# Autodesk Inventor assembly: Assieme
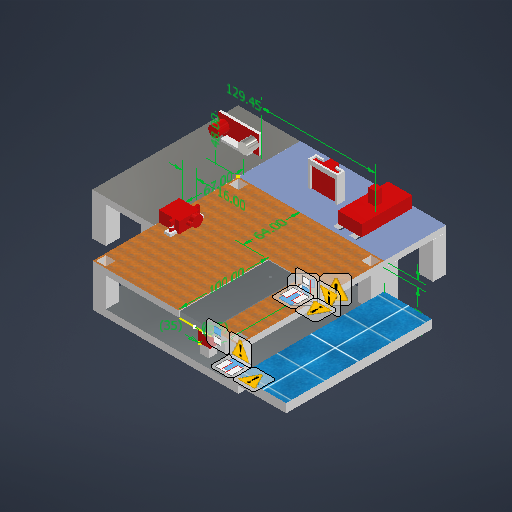
[picture p0: Inventor's stored thumbnail of the model, 512x512]
Saved by Autodesk Inventor 2026.2 (Build 302298000, 298)
## iProperties
Created: 2026-01-19
Part Number: Assieme
Document SubType Name: Assembly
Designer: ASUS
Mass: 649.981 g
Surface Area: 2252.42 cm^2
Volume: 649.981 cm^3
Density: 1 g/cm^3
Author: ASUS
## Documents named in this file (13)
- C:\Users\ASUS\Desktop\UNI\2 anno UNITN\EMBEDDED\Assieme.iam
- C:\Users\ASUS\Desktop\UNI\2 anno UNITN\EMBEDDED\cella di carico.ipt
- C:\Users\ASUS\Desktop\UNI\2 anno UNITN\EMBEDDED\distanziale cella di carico.ipt
- C:\Users\ASUS\Desktop\UNI\2 anno UNITN\EMBEDDED\piano di carico.ipt
- C:\Users\ASUS\Desktop\UNI\2 anno UNITN\EMBEDDED\piano inferiore.ipt
- C:\Users\ASUS\Desktop\UNI\2 anno UNITN\EMBEDDED\breadboard.ipt
- C:\Users\ASUS\Desktop\UNI\2 anno UNITN\EMBEDDED\piano superiore.ipt
- C:\Users\ASUS\Desktop\UNI\2 anno UNITN\EMBEDDED\Sensore ultrasuoni.ipt
- C:\Users\ASUS\Desktop\UNI\2 anno UNITN\EMBEDDED\Esp32.ipt
- C:\Users\ASUS\Desktop\UNI\2 anno UNITN\EMBEDDED\Micro servo.ipt
- C:\Users\ASUS\Desktop\UNI\2 anno UNITN\EMBEDDED\piano laterale.ipt
- C:\Users\ASUS\Desktop\UNI\2 anno UNITN\EMBEDDED\Schemo lcd.ipt
- C:\Users\ASUS\Desktop\UNI\2 anno UNITN\EMBEDDED\piano frontale.ipt
## Components (13 placed, 12 different names)
1. cella di carico:1 — Mate:1, Insert:1, Mate:2, Mate:3, Insert:2, Flush:1
2. distanziale cella di carico:1 — Mate:3, Insert:2, Mate:4, Insert:4
3. distanziale cella di carico:2 — Mate:1, Insert:1, Mate:2, Insert:3
4. piano di carico:1 — Insert:3, Flush:1, Flush:3
5. piano inferiore:1 — Mate:4, Mate:5, Insert:4, Flush:3, Mate:6, Flush:4, Mate:7, Flush:5, Flush:6, Flush:8
6. breadboard:1 — Mate:5, Mate:6, Flush:4
7. piano superiore:1 — Mate:7, Flush:5, Flush:6, Mate:8, Mate:9, Mate:10, Mate:11, Flush:7, Mate:12, Flush:10, Mate:16
8. Sensore ultrasuoni:1 — Mate:17, Mate:18
9. Esp32:1 — Mate:8, Mate:9
10. Micro servo:1 — Mate:10, Mate:11
11. piano laterale:1 — Flush:7, Flush:8, Mate:12, Mate:13, Mate:14, Mate:15, Flush:11
12. Schemo lcd:1 — Mate:13, Mate:14, Mate:15
13. piano frontale:1 — Flush:10, Mate:16, Flush:11, Mate:17, Mate:18
## Relationships (31: Mate 18, Flush 9, Insert 4)
- Mate:1: cella di carico:1 ↔ distanziale cella di carico:2
- Insert:1: cella di carico:1 ↔ distanziale cella di carico:2
- Mate:2: cella di carico:1 ↔ distanziale cella di carico:2
- Mate:3: cella di carico:1 ↔ distanziale cella di carico:1
- Insert:2: cella di carico:1 ↔ distanziale cella di carico:1
- Insert:3: distanziale cella di carico:2 ↔ piano di carico:1
- Flush:1: cella di carico:1 ↔ piano di carico:1
- Mate:4: distanziale cella di carico:1 ↔ piano inferiore:1
- Mate:5: piano inferiore:1 ↔ breadboard:1
- Insert:4: distanziale cella di carico:1 ↔ piano inferiore:1
- Flush:3: piano di carico:1 ↔ piano inferiore:1
- Mate:6: piano inferiore:1 ↔ breadboard:1
- Flush:4: piano inferiore:1 ↔ breadboard:1
- Mate:7: piano inferiore:1 ↔ piano superiore:1
- Flush:5: piano inferiore:1 ↔ piano superiore:1
- Flush:6: piano inferiore:1 ↔ piano superiore:1
- Mate:8: piano superiore:1 ↔ Esp32:1
- Mate:9 (10 mm): piano superiore:1 ↔ Esp32:1
- Mate:10: piano superiore:1 ↔ Micro servo:1
- Mate:11: piano superiore:1 ↔ Micro servo:1
- Flush:7: piano superiore:1 ↔ piano laterale:1
- Flush:8: piano inferiore:1 ↔ piano laterale:1
- Mate:12: piano superiore:1 ↔ piano laterale:1
- Mate:13: piano laterale:1 ↔ Schemo lcd:1
- Mate:14: piano laterale:1 ↔ Schemo lcd:1
- Mate:15 (2 mm): piano laterale:1 ↔ Schemo lcd:1
- Flush:10: piano superiore:1 ↔ piano frontale:1
- Mate:16: piano superiore:1 ↔ piano frontale:1
- Flush:11: piano laterale:1 ↔ piano frontale:1
- Mate:17: Sensore ultrasuoni:1 ↔ piano frontale:1
- Mate:18: Sensore ultrasuoni:1 ↔ piano frontale:1
## Named parameters: Finish1_Area = 89.1, Finish2_Area = 263.17, Finish3_Area = 17.92, Finish3_Thickness = 0.05 mm, Finish4_Area = 101.676, Finish4_Thickness = 0.05 mm, Finish5_Area = 13.0529, Finish5_Thickness = 0.05 mm, Finish6_Area = 117.555, Finish6_Thickness = 0.05 mm, Finish7_Area = 104.64, Finish7_Thickness = 0.05 mm, Finish8_Area = 229.36, Finish8_Thickness = 0.05 mm
note: some values were not read from the file. Shown as the stored number, unit unknown: "Finish1_Area", "Finish2_Area", "Finish3_Area", "Finish4_Area", "Finish5_Area", "Finish6_Area", "Finish7_Area", "Finish8_Area".
